# Autodesk Inventor assembly: Drive Arm
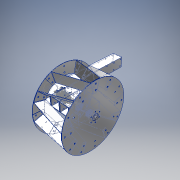
[picture p0: Inventor's stored thumbnail of the model, 180x180]
Saved by Autodesk Inventor 2019 (Build 230136000, 136)
## iProperties
Created: 2018-10-29
Part Number: Drive Arm
Document SubType Name: Assembly
Designer: Adhik
Author: Adhik
## Documents named in this file (11)
- I:\CAD\Julie\Drive Arm.iam
- I:\CAD\Julie\Arm 18 inch.ipt
- I:\CAD\Julie\Arm 2 inch A.ipt
- I:\CAD\Julie\Arm 2 inch B.ipt
- I:\CAD\Julie\Arm 2 inch C.ipt
- I:\CAD\Julie\Arm Bearing.ipt
- I:\CAD\Julie\Gearbox.ipt
- I:\CAD\Julie\Shaft.ipt
- I:\CAD\Julie\Shaft Coupler.ipt
- I:\CAD\Julie\Wheel.iam
- I:\CAD\Julie\3775.ipt
## Components (11 placed, 10 different names)
1. Arm 18 inch:1 — Flush:1, Flush:4, Mate:3
2. Arm 2 inch A:1 — Flush:1, Flush:2, Flush:4, Flush:5, Mate:2, Mate:3, Mate:4, Mate:15
3. Arm 2 inch B:1 — Flush:2, Flush:3, Flush:5, Flush:6, Mate:1, Mate:2, Insert:1, Mate:16
4. Arm 2 inch C:1 — Flush:3, Flush:6, Mate:1, Insert:2
5. Arm Bearing:1 — Insert:1, Mate:10
6. Arm Bearing:2 — Insert:2, Mate:7, Mate:12
7. Gearbox:1 — Mate:4, Mate:8, Mate:9, Mate:13, Mate:14, Mate:15, Mate:16
8. Shaft:1 — Mate:7, Mate:8, Mate:11
9. Shaft Coupler:1 — Mate:9, Mate:10
10. Wheel:1 [sub-assembly] — Mate:11, Mate:12
11. 3775:1 — Mate:13, Mate:14
## Relationships (22: Mate 14, Flush 6, Insert 2)
- Flush:1: Arm 18 inch:1 ↔ Arm 2 inch A:1
- Flush:2: Arm 2 inch A:1 ↔ Arm 2 inch B:1
- Flush:3: Arm 2 inch B:1 ↔ Arm 2 inch C:1
- Flush:4: Arm 18 inch:1 ↔ Arm 2 inch A:1
- Flush:5: Arm 2 inch A:1 ↔ Arm 2 inch B:1
- Flush:6: Arm 2 inch B:1 ↔ Arm 2 inch C:1
- Mate:1: Arm 2 inch B:1 ↔ Arm 2 inch C:1
- Mate:2: Arm 2 inch A:1 ↔ Arm 2 inch B:1
- Mate:3: Arm 18 inch:1 ↔ Arm 2 inch A:1
- Insert:1: Arm 2 inch B:1 ↔ Arm Bearing:1
- Insert:2: Arm 2 inch C:1 ↔ Arm Bearing:2
- Mate:4: Arm 2 inch A:1 ↔ Gearbox:1
- Mate:7: Arm Bearing:2 ↔ Shaft:1
- Mate:8: Gearbox:1 ↔ Shaft:1
- Mate:9: Gearbox:1 ↔ Shaft Coupler:1
- Mate:10: Arm Bearing:1 ↔ Shaft Coupler:1
- Mate:11: Shaft:1 ↔ Wheel:1
- Mate:12: Arm Bearing:2 ↔ Wheel:1
- Mate:13: Gearbox:1 ↔ 3775:1
- Mate:14: Gearbox:1 ↔ 3775:1
- Mate:15: Arm 2 inch A:1 ↔ Gearbox:1
- Mate:16: Arm 2 inch B:1 ↔ Gearbox:1
